# Autodesk Inventor assembly: Box Arm
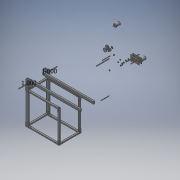
[picture p0: Inventor's stored thumbnail of the model, 180x180]
Saved by Autodesk Inventor 2018 (Build 220112000, 112)
## iProperties
Created: 2019-01-16
Part Number: Box Arm
Document SubType Name: Assembly
Designer: Gabriel
Author: Gabriel
## Documents named in this file (29)
- C:\Users\Gabriel\Documents\GitHub\2019CAD\Drivebase Box Arm\Box Arm.iam
- C:\Users\Gabriel\Documents\GitHub\2019CAD\Drivebase Box Arm\30in 1x1 Beam.ipt
- C:\Users\Gabriel\Documents\GitHub\2019CAD\Drivebase Box Arm\25in 1x1 Beam.ipt
- C:\Users\Gabriel\Documents\GitHub\2019CAD\Drivebase Box Arm\17in 1x1 Beam.ipt
- C:\Users\Gabriel\Documents\GitHub\2019CAD\Drivebase Box Arm\23in 1x1 Beam.ipt
- C:\Users\Gabriel\Documents\GitHub\2019CAD\Drivebase Box Arm\L gusset.ipt
- C:\Users\Gabriel\Documents\GitHub\2019CAD\Drivebase Box Arm\34.48in Arm Bea.ipt
- C:\Users\Gabriel\Documents\GitHub\2019CAD\Drivebase Box Arm\0_500_ID_x_1_125_OD_x_0_313_WD_Flanged_Bearing_217-2731.ipt
- C:\Users\Gabriel\Documents\GitHub\2019CAD\Drivebase Box Arm\_72t_Aluminum_Plate_Sprocket_25_Chain_1-1_8_Bearing_Bore_217-2627.ipt
- C:\Users\Gabriel\Documents\GitHub\2019CAD\Drivebase Box Arm\Hex Hub.ipt
- C:\Users\Gabriel\Documents\GitHub\2019CAD\Drivebase Box Arm\0.5in Hex Shaft.ipt
- C:\Users\Gabriel\Documents\GitHub\2019CAD\Drivebase Box Arm\half_inch_collar.ipt
- C:\Users\Gabriel\Documents\GitHub\2019CAD\Drivebase Box Arm\1_2_Acetal_Spacer_-_1_2_Hex_217-3261.ipt
- C:\Users\Gabriel\Documents\GitHub\2019CAD\Drivebase Box Arm\am-0150 Toughbox Large Output Gear.ipt
- C:\Users\Gabriel\Documents\GitHub\2019CAD\Drivebase Box Arm\Mini_CIM_Motor_217-3371.ipt
- C:\Users\Gabriel\Documents\GitHub\2019CAD\Drivebase Box Arm\ARm Gearbox Plate.ipt
- C:\Users\Gabriel\Documents\GitHub\2019CAD\Drivebase Box Arm\1_16_Acetal_Spacer_-_1_2_Hex_217-3257.ipt
- C:\Users\Gabriel\Documents\GitHub\2019CAD\Drivebase Box Arm\3_8in Hex Shaft.ipt
- C:\Users\Gabriel\Documents\GitHub\2019CAD\Drivebase Box Arm\10T_Steel_Spur_Gear_20_DP_12T_Center_Distance_CIM_Motor_217-6334.ipt
- C:\Users\Gabriel\Documents\GitHub\2019CAD\Drivebase Box Arm\am-0143 50 Tooth 20 dp Aluminum Gear 375 Hex.ipt
- C:\Users\Gabriel\Documents\GitHub\2019CAD\Drivebase Box Arm\am-0151 14T 20dp 375hex.ipt
- C:\Users\Gabriel\Documents\GitHub\2019CAD\Drivebase Box Arm\1_16_Acetal_Spacer_-_3_8_Hex_217-3258.ipt
- C:\Users\Gabriel\Documents\GitHub\2019CAD\Drivebase Box Arm\40t_Aluminum_Spur_Gear_20_DP_3_8_Hex_Bore_217-2707.ipt
- C:\Users\Gabriel\Documents\GitHub\2019CAD\Drivebase Box Arm\am-0028 00.375'' id Flanged, Shielded Ball Bearing (FR6ZZ).ipt
- C:\Users\Gabriel\Documents\GitHub\2019CAD\Drivebase Box Arm\USS flat washer #10 2993.ipt
- C:\Users\Gabriel\Documents\GitHub\2019CAD\Drivebase Box Arm\92196A271_18-8 STAINLESS STEEL SOCKET HEAD CAP SCREW.ipt
- C:\Users\Gabriel\Documents\GitHub\2019CAD\Drivebase Box Arm\am-3621 - S25-18HA-500H.ipt
- C:\Users\Gabriel\Downloads\Clamping_Shaft_Collar_-_1_2_Hex_ID_217-2737.ipt
- C:\Users\Gabriel\Downloads\Clamping_Shaft_Collar_-_3_8_Hex_ID_217-2739.ipt
## Components (108 placed, 28 different names)
1. 30in 1x1 Beam:1 — Mate:13, Mate:14, Mate:37, Mate:38, Mate:74, Mate:75, Mate:83, Mate:84, Mate:98, Mate:99, Mate:101, Mate:102, Mate:103, Mate:104
2. 30in 1x1 Beam:2 — Mate:11, Mate:12, Mate:39, Mate:40, Mate:73, Mate:76, Mate:86, Mate:87, Mate:95, Mate:96, Mate:105, Mate:106, Mate:107, Mate:108
3. 25in 1x1 Beam:1 — Mate:57, Mate:58, Mate:59, Mate:60, Mate:65, Mate:66, Mate:90, Mate:91
4. 25in 1x1 Beam:2 — Mate:61, Mate:62, Mate:63, Mate:64, Mate:67, Mate:68, Mate:93, Mate:94
5. 25in 1x1 Beam:3 — Mate:29, Mate:30, Mate:53, Mate:54, Mate:97
6. 25in 1x1 Beam:4 — Mate:31, Mate:32, Mate:55, Mate:56, Mate:100
7. 17in 1x1 Beam:1 — Mate:69, Mate:70, Mate:71, Mate:72
8. 17in 1x1 Beam:2 — Mate:21, Mate:22, Mate:23, Mate:24
9. 23in 1x1 Beam:1 — Mate:43, Mate:44, Mate:49, Mate:50, Mate:88, Mate:92
10. 23in 1x1 Beam:2 — Mate:47, Mate:48, Mate:51, Mate:52, Mate:85, Mate:89
11. L gusset:1 — Mate:53, Mate:54, Mate:63, Mate:64
12. L gusset:4 — Mate:49, Mate:50, Mate:61, Mate:62
13. L gusset:5 — Mate:51, Mate:52, Mate:57, Mate:58
14. L gusset:7 — Mate:11, Mate:12, Mate:23, Mate:24
15. L gusset:9 — Mate:13, Mate:14, Mate:21, Mate:22
16. L gusset:11 — Mate:31, Mate:32, Mate:74, Mate:75
17. L gusset:12 — Mate:29, Mate:30, Mate:73, Mate:76
18. L gusset:13 — Mate:43, Mate:44
19. L gusset:14 — Mate:47, Mate:48
20. L gusset:15 — Mate:39, Mate:40, Mate:77, Mate:80
21. L gusset:16 — Mate:37, Mate:38, Mate:78, Mate:79
22. L gusset:17 — Mate:55, Mate:56, Mate:59, Mate:60
23. L gusset:18 — Mate:67, Mate:68, Mate:69, Mate:70
24. L gusset:19 — Mate:65, Mate:66, Mate:71, Mate:72
25. 17in 1x1 Beam:3 — Mate:77, Mate:78, Mate:79, Mate:80
26. 34.48in Arm Bea:2 — Mate:109, Mate:110
27. 0_500_ID_x_1_125_OD_x_0_313_WD_Flanged_Bearing_217-2731:1 — Mate:103, Mate:104, Mate:139, Mate:140, Mate:149
28. 0_500_ID_x_1_125_OD_x_0_313_WD_Flanged_Bearing_217-2731:2 — Mate:107, Mate:108, Mate:126, Mate:152
29. 0_500_ID_x_1_125_OD_x_0_313_WD_Flanged_Bearing_217-2731:5 — Mate:101, Mate:102, Mate:143
30. 0_500_ID_x_1_125_OD_x_0_313_WD_Flanged_Bearing_217-2731:8 — Mate:105, Mate:106, Mate:122
31. L gusset:20 — Mate:92, Mate:93, Mate:94
32. L gusset:21 — Mate:89, Mate:90, Mate:91
33. L gusset:22 — Mate:98, Mate:99, Mate:100
34. L gusset:23 — Mate:95, Mate:96, Mate:97
35. L gusset:24 — Mate:83, Mate:84, Mate:85
36. L gusset:25 — Mate:86, Mate:87, Mate:88
37. _72t_Aluminum_Plate_Sprocket_25_Chain_1-1_8_Bearing_Bore_217-2627:2 — Mate:120, Mate:121, Mate:138
38. Hex Hub:2 — Mate:109, Mate:110, Mate:111, Mate:112, Mate:113, Mate:114, Mate:115
39. Hex Hub:3 — Mate:116, Mate:117, Mate:118, Mate:120, Mate:121, Mate:122, Mate:138
40. 0.5in Hex Shaft:2 — Mate:114, Mate:115, Mate:116, Mate:117, Mate:123, Mate:124, Mate:125, Mate:150, Mate:151, Mate:404, Mate:405
41. 1_2_Acetal_Spacer_-_1_2_Hex_217-3261:1 — Mate:123, Mate:124, Mate:125, Mate:126, Mate:406
42. 1_2_Acetal_Spacer_-_1_2_Hex_217-3261:3 — Mate:111, Mate:112, Mate:113, Mate:118
43. 34.48in Arm Bea:3 — Mate:128
44. _72t_Aluminum_Plate_Sprocket_25_Chain_1-1_8_Bearing_Bore_217-2627:3 — Mate:137
45. Hex Hub:4 — Mate:134, Mate:135, Mate:136, Mate:137, Mate:139, Mate:140
46. Hex Hub:5 — Mate:128, Mate:129, Mate:130, Mate:133
47. 0.5in Hex Shaft:3 — Mate:129, Mate:130, Mate:131, Mate:132, Mate:134, Mate:135, Mate:141, Mate:142, Mate:147, Mate:148, Mate:401, Mate:402
48. 1_2_Acetal_Spacer_-_1_2_Hex_217-3261:7 — Mate:141, Mate:142, Mate:143, Mate:403
49. 1_2_Acetal_Spacer_-_1_2_Hex_217-3261:8 — Mate:131, Mate:132, Mate:133, Mate:136
50. 1_2_Acetal_Spacer_-_1_2_Hex_217-3261:9 — Mate:147, Mate:148, Mate:149
51. 1_2_Acetal_Spacer_-_1_2_Hex_217-3261:10 — Mate:150, Mate:151, Mate:152
52. 0.5in Hex Shaft:4
53. 0.5in Hex Shaft:5 — Mate:345, Mate:346, Mate:347, Mate:348, Mate:349, Mate:350, Mate:351, Mate:370, Mate:371, Mate:386, Mate:387, Mate:389, Mate:390, Mate:395, Mate:396, Mate:398, Mate:399
54. half_inch_collar:9
55. Mini_CIM_Motor_217-3371:5 — Mate:368, Mate:369, Mate:374
56. am-0150 Toughbox Large Output Gear:8 — Mate:345, Mate:346, Mate:347, Mate:352
57. Mini_CIM_Motor_217-3371:8
58. 1_16_Acetal_Spacer_-_1_2_Hex_217-3257:4 — Mate:348, Mate:349, Mate:352, Mate:353
59. 1_16_Acetal_Spacer_-_1_2_Hex_217-3257:6 — Mate:350, Mate:351, Mate:353, Mate:354
60. 1_16_Acetal_Spacer_-_1_2_Hex_217-3257:8 — Mate:370, Mate:371, Mate:372, Mate:388
61. 3_8in Hex Shaft:2
62. 3_8in Hex Shaft:5 — Mate:313, Mate:314, Mate:315, Mate:316, Mate:317, Mate:318, Mate:321, Mate:322, Mate:357, Mate:358, Mate:394
63. am-0151 14T 20dp 375hex:1 — Mate:325, Mate:326, Mate:331, Mate:335
64. am-0151 14T 20dp 375hex:3 — Mate:315, Mate:316, Mate:320, Mate:359
65. 10T_Steel_Spur_Gear_20_DP_12T_Center_Distance_CIM_Motor_217-6334:4
66. am-0151 14T 20dp 375hex:4
67. am-0143 50 Tooth 20 dp Aluminum Gear 375 Hex:5 — Mate:327, Mate:328, Mate:332, Mate:339
68. 10T_Steel_Spur_Gear_20_DP_12T_Center_Distance_CIM_Motor_217-6334:6 — Mate:374
69. am-0143 50 Tooth 20 dp Aluminum Gear 375 Hex:6
70. am-0151 14T 20dp 375hex:6
71. 1_16_Acetal_Spacer_-_3_8_Hex_217-3258:2 — Mate:337, Mate:338, Mate:339
72. 1_16_Acetal_Spacer_-_3_8_Hex_217-3258:3 — Mate:333, Mate:334, Mate:335, Mate:384
73. 1_16_Acetal_Spacer_-_3_8_Hex_217-3258:5 — Mate:321, Mate:322, Mate:323
74. 1_16_Acetal_Spacer_-_3_8_Hex_217-3258:6 — Mate:317, Mate:318, Mate:319, Mate:320
75. 40t_Aluminum_Spur_Gear_20_DP_3_8_Hex_Bore_217-2707:1 — Mate:313, Mate:314, Mate:319, Mate:323
76. 40t_Aluminum_Spur_Gear_20_DP_3_8_Hex_Bore_217-2707:3
77. 3_8in Hex Shaft:8
78. 3_8in Hex Shaft:10 — Mate:325, Mate:326, Mate:327, Mate:328, Mate:329, Mate:330, Mate:333, Mate:334, Mate:337, Mate:338
79. ARm Gearbox Plate:5 — Mate:341, Mate:344, Mate:378, Mate:379, Mate:382, Mate:383
80. ARm Gearbox Plate:6 — Mate:342, Mate:343, Mate:360, Mate:361, Mate:362, Mate:363, Mate:365, Mate:367, Mate:376, Mate:377, Mate:380, Mate:381
81. 1_16_Acetal_Spacer_-_3_8_Hex_217-3258:8 — Mate:357, Mate:358, Mate:359
82. 1_16_Acetal_Spacer_-_3_8_Hex_217-3258:10 — Mate:329, Mate:330, Mate:331, Mate:332
83. 0_500_ID_x_1_125_OD_x_0_313_WD_Flanged_Bearing_217-2731:9 — Mate:341, Mate:344, Mate:400
84. 0_500_ID_x_1_125_OD_x_0_313_WD_Flanged_Bearing_217-2731:10 — Mate:342, Mate:343, Mate:354, Mate:372
85. USS flat washer #10 2993:1 — Mate:366, Mate:367, Mate:369
86. USS flat washer #10 2993:2 — Mate:364, Mate:365
87. 92196A271_18-8 STAINLESS STEEL SOCKET HEAD CAP SCREW:1 — Mate:361, Mate:363, Mate:366
88. 92196A271_18-8 STAINLESS STEEL SOCKET HEAD CAP SCREW:2 — Mate:360, Mate:362, Mate:364, Mate:368
89. am-0028 00.375'' id Flanged, Shielded Ball Bearing (FR6ZZ):2 — Mate:376, Mate:380, Mate:384
90. am-0028 00.375'' id Flanged, Shielded Ball Bearing (FR6ZZ):3 — Mate:378, Mate:383
91. am-0028 00.375'' id Flanged, Shielded Ball Bearing (FR6ZZ):4 — Mate:379, Mate:382
92. am-0028 00.375'' id Flanged, Shielded Ball Bearing (FR6ZZ):5 — Mate:377, Mate:381, Mate:394
93. am-0150 Toughbox Large Output Gear:9
94. am-3621 - S25-18HA-500H:1 — Mate:386, Mate:387, Mate:388, Mate:391
95. 1_2_Acetal_Spacer_-_1_2_Hex_217-3261:11 — Mate:389, Mate:390, Mate:391, Mate:397
96. am-3621 - S25-18HA-500H:2
97. Clamping_Shaft_Collar_-_1_2_Hex_ID_217-2737:1 — Mate:395, Mate:396, Mate:397
98. Clamping_Shaft_Collar_-_3_8_Hex_ID_217-2739:1
99. Clamping_Shaft_Collar_-_1_2_Hex_ID_217-2737:2 — Mate:398, Mate:399, Mate:400
100. Clamping_Shaft_Collar_-_3_8_Hex_ID_217-2739:2
101. Clamping_Shaft_Collar_-_1_2_Hex_ID_217-2737:3
102. Clamping_Shaft_Collar_-_3_8_Hex_ID_217-2739:3
103. Clamping_Shaft_Collar_-_1_2_Hex_ID_217-2737:4
104. Clamping_Shaft_Collar_-_3_8_Hex_ID_217-2739:4
105. Clamping_Shaft_Collar_-_1_2_Hex_ID_217-2737:5 — Mate:404, Mate:405, Mate:406
106. Clamping_Shaft_Collar_-_3_8_Hex_ID_217-2739:5
107. Clamping_Shaft_Collar_-_1_2_Hex_ID_217-2737:6 — Mate:401, Mate:402, Mate:403
108. Clamping_Shaft_Collar_-_3_8_Hex_ID_217-2739:6
## Relationships (201: Mate 201)
- Mate:11: 30in 1x1 Beam:2 ↔ L gusset:7
- Mate:12: 30in 1x1 Beam:2 ↔ L gusset:7
- Mate:13: 30in 1x1 Beam:1 ↔ L gusset:9
- Mate:14: 30in 1x1 Beam:1 ↔ L gusset:9
- Mate:21: 17in 1x1 Beam:2 ↔ L gusset:9
- Mate:22: 17in 1x1 Beam:2 ↔ L gusset:9
- Mate:23: 17in 1x1 Beam:2 ↔ L gusset:7
- Mate:24: 17in 1x1 Beam:2 ↔ L gusset:7
- Mate:29: 25in 1x1 Beam:3 ↔ L gusset:12
- Mate:30: 25in 1x1 Beam:3 ↔ L gusset:12
- Mate:31: 25in 1x1 Beam:4 ↔ L gusset:11
- Mate:32: 25in 1x1 Beam:4 ↔ L gusset:11
- Mate:37: 30in 1x1 Beam:1 ↔ L gusset:16
- Mate:38: 30in 1x1 Beam:1 ↔ L gusset:16
- Mate:39: 30in 1x1 Beam:2 ↔ L gusset:15
- Mate:40: 30in 1x1 Beam:2 ↔ L gusset:15
- Mate:43: 23in 1x1 Beam:1 ↔ L gusset:13
- Mate:44: 23in 1x1 Beam:1 ↔ L gusset:13
- Mate:47: 23in 1x1 Beam:2 ↔ L gusset:14
- Mate:48: 23in 1x1 Beam:2 ↔ L gusset:14
- Mate:49: 23in 1x1 Beam:1 ↔ L gusset:4
- Mate:50: 23in 1x1 Beam:1 ↔ L gusset:4
- Mate:51: 23in 1x1 Beam:2 ↔ L gusset:5
- Mate:52: 23in 1x1 Beam:2 ↔ L gusset:5
- Mate:53: 25in 1x1 Beam:3 ↔ L gusset:1
- Mate:54: 25in 1x1 Beam:3 ↔ L gusset:1
- Mate:55: 25in 1x1 Beam:4 ↔ L gusset:17
- Mate:56: 25in 1x1 Beam:4 ↔ L gusset:17
- Mate:57: 25in 1x1 Beam:1 ↔ L gusset:5
- Mate:58: 25in 1x1 Beam:1 ↔ L gusset:5
- Mate:59: 25in 1x1 Beam:1 ↔ L gusset:17
- Mate:60: 25in 1x1 Beam:1 ↔ L gusset:17
- Mate:61: 25in 1x1 Beam:2 ↔ L gusset:4
- Mate:62: 25in 1x1 Beam:2 ↔ L gusset:4
- Mate:63: 25in 1x1 Beam:2 ↔ L gusset:1
- Mate:64: 25in 1x1 Beam:2 ↔ L gusset:1
- Mate:65: 25in 1x1 Beam:1 ↔ L gusset:19
- Mate:66: 25in 1x1 Beam:1 ↔ L gusset:19
- Mate:67: 25in 1x1 Beam:2 ↔ L gusset:18
- Mate:68: 25in 1x1 Beam:2 ↔ L gusset:18
- Mate:69: 17in 1x1 Beam:1 ↔ L gusset:18
- Mate:70: 17in 1x1 Beam:1 ↔ L gusset:18
- Mate:71: 17in 1x1 Beam:1 ↔ L gusset:19
- Mate:72: 17in 1x1 Beam:1 ↔ L gusset:19
- Mate:73: 30in 1x1 Beam:2 ↔ L gusset:12
- Mate:74: 30in 1x1 Beam:1 ↔ L gusset:11
- Mate:75: 30in 1x1 Beam:1 ↔ L gusset:11
- Mate:76: 30in 1x1 Beam:2 ↔ L gusset:12
- Mate:77: L gusset:15 ↔ 17in 1x1 Beam:3
- Mate:78: L gusset:16 ↔ 17in 1x1 Beam:3
- Mate:79: L gusset:16 ↔ 17in 1x1 Beam:3
- Mate:80: L gusset:15 ↔ 17in 1x1 Beam:3
- Mate:83: 30in 1x1 Beam:1 ↔ L gusset:24
- Mate:84: 30in 1x1 Beam:1 ↔ L gusset:24
- Mate:85: 23in 1x1 Beam:2 ↔ L gusset:24
- Mate:86: 30in 1x1 Beam:2 ↔ L gusset:25
- Mate:87: 30in 1x1 Beam:2 ↔ L gusset:25
- Mate:88: 23in 1x1 Beam:1 ↔ L gusset:25
- Mate:89: 23in 1x1 Beam:2 ↔ L gusset:21
- Mate:90: 25in 1x1 Beam:1 ↔ L gusset:21
- Mate:91: 25in 1x1 Beam:1 ↔ L gusset:21
- Mate:92: 23in 1x1 Beam:1 ↔ L gusset:20
- Mate:93: 25in 1x1 Beam:2 ↔ L gusset:20
- Mate:94: 25in 1x1 Beam:2 ↔ L gusset:20
- Mate:95: 30in 1x1 Beam:2 ↔ L gusset:23
- Mate:96: 30in 1x1 Beam:2 ↔ L gusset:23
- Mate:97: 25in 1x1 Beam:3 ↔ L gusset:23
- Mate:98: 30in 1x1 Beam:1 ↔ L gusset:22
- Mate:99: 30in 1x1 Beam:1 ↔ L gusset:22
- Mate:100: 25in 1x1 Beam:4 ↔ L gusset:22
- Mate:101: 30in 1x1 Beam:1 ↔ 0_500_ID_x_1_125_OD_x_0_313_WD_Flanged_Bearing_217-2731:5
- Mate:102: 30in 1x1 Beam:1 ↔ 0_500_ID_x_1_125_OD_x_0_313_WD_Flanged_Bearing_217-2731:5
- Mate:103: 30in 1x1 Beam:1 ↔ 0_500_ID_x_1_125_OD_x_0_313_WD_Flanged_Bearing_217-2731:1
- Mate:104: 30in 1x1 Beam:1 ↔ 0_500_ID_x_1_125_OD_x_0_313_WD_Flanged_Bearing_217-2731:1
- Mate:105: 30in 1x1 Beam:2 ↔ 0_500_ID_x_1_125_OD_x_0_313_WD_Flanged_Bearing_217-2731:8
- Mate:106: 30in 1x1 Beam:2 ↔ 0_500_ID_x_1_125_OD_x_0_313_WD_Flanged_Bearing_217-2731:8
- Mate:107: 30in 1x1 Beam:2 ↔ 0_500_ID_x_1_125_OD_x_0_313_WD_Flanged_Bearing_217-2731:2
- Mate:108: 30in 1x1 Beam:2 ↔ 0_500_ID_x_1_125_OD_x_0_313_WD_Flanged_Bearing_217-2731:2
- Mate:109: 34.48in Arm Bea:2 ↔ Hex Hub:2
- Mate:110: 34.48in Arm Bea:2 ↔ Hex Hub:2
- Mate:111: Hex Hub:2 ↔ 1_2_Acetal_Spacer_-_1_2_Hex_217-3261:3
- Mate:112: Hex Hub:2 ↔ 1_2_Acetal_Spacer_-_1_2_Hex_217-3261:3
- Mate:113: Hex Hub:2 ↔ 1_2_Acetal_Spacer_-_1_2_Hex_217-3261:3
- Mate:114: Hex Hub:2 ↔ 0.5in Hex Shaft:2
- Mate:115: Hex Hub:2 ↔ 0.5in Hex Shaft:2
- Mate:116: Hex Hub:3 ↔ 0.5in Hex Shaft:2
- Mate:117: Hex Hub:3 ↔ 0.5in Hex Shaft:2
- Mate:118: Hex Hub:3 ↔ 1_2_Acetal_Spacer_-_1_2_Hex_217-3261:3
- Mate:120: _72t_Aluminum_Plate_Sprocket_25_Chain_1-1_8_Bearing_Bore_217-2627:2 ↔ Hex Hub:3
- Mate:121: _72t_Aluminum_Plate_Sprocket_25_Chain_1-1_8_Bearing_Bore_217-2627:2 ↔ Hex Hub:3
- Mate:122: 0_500_ID_x_1_125_OD_x_0_313_WD_Flanged_Bearing_217-2731:8 ↔ Hex Hub:3
- Mate:123: 0.5in Hex Shaft:2 ↔ 1_2_Acetal_Spacer_-_1_2_Hex_217-3261:1
- Mate:124: 0.5in Hex Shaft:2 ↔ 1_2_Acetal_Spacer_-_1_2_Hex_217-3261:1
- Mate:125: 0.5in Hex Shaft:2 ↔ 1_2_Acetal_Spacer_-_1_2_Hex_217-3261:1
- Mate:126: 0_500_ID_x_1_125_OD_x_0_313_WD_Flanged_Bearing_217-2731:2 ↔ 1_2_Acetal_Spacer_-_1_2_Hex_217-3261:1
- Mate:128: 34.48in Arm Bea:3 ↔ Hex Hub:5
- Mate:129: Hex Hub:5 ↔ 0.5in Hex Shaft:3
- Mate:130: Hex Hub:5 ↔ 0.5in Hex Shaft:3
- Mate:131: 0.5in Hex Shaft:3 ↔ 1_2_Acetal_Spacer_-_1_2_Hex_217-3261:8
- Mate:132: 0.5in Hex Shaft:3 ↔ 1_2_Acetal_Spacer_-_1_2_Hex_217-3261:8
- Mate:133: Hex Hub:5 ↔ 1_2_Acetal_Spacer_-_1_2_Hex_217-3261:8
- Mate:134: Hex Hub:4 ↔ 0.5in Hex Shaft:3
- Mate:135: Hex Hub:4 ↔ 0.5in Hex Shaft:3
- Mate:136: Hex Hub:4 ↔ 1_2_Acetal_Spacer_-_1_2_Hex_217-3261:8
- Mate:137: _72t_Aluminum_Plate_Sprocket_25_Chain_1-1_8_Bearing_Bore_217-2627:3 ↔ Hex Hub:4
- Mate:138: _72t_Aluminum_Plate_Sprocket_25_Chain_1-1_8_Bearing_Bore_217-2627:2 ↔ Hex Hub:3
- Mate:139: 0_500_ID_x_1_125_OD_x_0_313_WD_Flanged_Bearing_217-2731:1 ↔ Hex Hub:4
- Mate:140: 0_500_ID_x_1_125_OD_x_0_313_WD_Flanged_Bearing_217-2731:1 ↔ Hex Hub:4
- Mate:141: 0.5in Hex Shaft:3 ↔ 1_2_Acetal_Spacer_-_1_2_Hex_217-3261:7
- Mate:142: 0.5in Hex Shaft:3 ↔ 1_2_Acetal_Spacer_-_1_2_Hex_217-3261:7
- Mate:143: 0_500_ID_x_1_125_OD_x_0_313_WD_Flanged_Bearing_217-2731:5 ↔ 1_2_Acetal_Spacer_-_1_2_Hex_217-3261:7
- Mate:147: 0.5in Hex Shaft:3 ↔ 1_2_Acetal_Spacer_-_1_2_Hex_217-3261:9
- Mate:148: 0.5in Hex Shaft:3 ↔ 1_2_Acetal_Spacer_-_1_2_Hex_217-3261:9
- Mate:149: 0_500_ID_x_1_125_OD_x_0_313_WD_Flanged_Bearing_217-2731:1 ↔ 1_2_Acetal_Spacer_-_1_2_Hex_217-3261:9
- Mate:150: 0.5in Hex Shaft:2 ↔ 1_2_Acetal_Spacer_-_1_2_Hex_217-3261:10
- Mate:151: 0.5in Hex Shaft:2 ↔ 1_2_Acetal_Spacer_-_1_2_Hex_217-3261:10
- Mate:152: 0_500_ID_x_1_125_OD_x_0_313_WD_Flanged_Bearing_217-2731:2 ↔ 1_2_Acetal_Spacer_-_1_2_Hex_217-3261:10
- Mate:313: 3_8in Hex Shaft:5 ↔ 40t_Aluminum_Spur_Gear_20_DP_3_8_Hex_Bore_217-2707:1
- Mate:314: 3_8in Hex Shaft:5 ↔ 40t_Aluminum_Spur_Gear_20_DP_3_8_Hex_Bore_217-2707:1
- Mate:315: 3_8in Hex Shaft:5 ↔ am-0151 14T 20dp 375hex:3
- Mate:316: 3_8in Hex Shaft:5 ↔ am-0151 14T 20dp 375hex:3
- Mate:317: 3_8in Hex Shaft:5 ↔ 1_16_Acetal_Spacer_-_3_8_Hex_217-3258:6
- Mate:318: 3_8in Hex Shaft:5 ↔ 1_16_Acetal_Spacer_-_3_8_Hex_217-3258:6
- Mate:319: 1_16_Acetal_Spacer_-_3_8_Hex_217-3258:6 ↔ 40t_Aluminum_Spur_Gear_20_DP_3_8_Hex_Bore_217-2707:1
- Mate:320: am-0151 14T 20dp 375hex:3 ↔ 1_16_Acetal_Spacer_-_3_8_Hex_217-3258:6
- Mate:321: 3_8in Hex Shaft:5 ↔ 1_16_Acetal_Spacer_-_3_8_Hex_217-3258:5
- Mate:322: 3_8in Hex Shaft:5 ↔ 1_16_Acetal_Spacer_-_3_8_Hex_217-3258:5
- Mate:323: 1_16_Acetal_Spacer_-_3_8_Hex_217-3258:5 ↔ 40t_Aluminum_Spur_Gear_20_DP_3_8_Hex_Bore_217-2707:1
- Mate:325: am-0151 14T 20dp 375hex:1 ↔ 3_8in Hex Shaft:10
- Mate:326: am-0151 14T 20dp 375hex:1 ↔ 3_8in Hex Shaft:10
- Mate:327: am-0143 50 Tooth 20 dp Aluminum Gear 375 Hex:5 ↔ 3_8in Hex Shaft:10
- Mate:328: am-0143 50 Tooth 20 dp Aluminum Gear 375 Hex:5 ↔ 3_8in Hex Shaft:10
- Mate:329: 3_8in Hex Shaft:10 ↔ 1_16_Acetal_Spacer_-_3_8_Hex_217-3258:10
- Mate:330: 3_8in Hex Shaft:10 ↔ 1_16_Acetal_Spacer_-_3_8_Hex_217-3258:10
- Mate:331: am-0151 14T 20dp 375hex:1 ↔ 1_16_Acetal_Spacer_-_3_8_Hex_217-3258:10
- Mate:332: am-0143 50 Tooth 20 dp Aluminum Gear 375 Hex:5 ↔ 1_16_Acetal_Spacer_-_3_8_Hex_217-3258:10
- Mate:333: 1_16_Acetal_Spacer_-_3_8_Hex_217-3258:3 ↔ 3_8in Hex Shaft:10
- Mate:334: 1_16_Acetal_Spacer_-_3_8_Hex_217-3258:3 ↔ 3_8in Hex Shaft:10
- Mate:335: am-0151 14T 20dp 375hex:1 ↔ 1_16_Acetal_Spacer_-_3_8_Hex_217-3258:3
- Mate:337: 1_16_Acetal_Spacer_-_3_8_Hex_217-3258:2 ↔ 3_8in Hex Shaft:10
- Mate:338: 1_16_Acetal_Spacer_-_3_8_Hex_217-3258:2 ↔ 3_8in Hex Shaft:10
- Mate:339: am-0143 50 Tooth 20 dp Aluminum Gear 375 Hex:5 ↔ 1_16_Acetal_Spacer_-_3_8_Hex_217-3258:2
- Mate:341: ARm Gearbox Plate:5 ↔ 0_500_ID_x_1_125_OD_x_0_313_WD_Flanged_Bearing_217-2731:9
- Mate:342: ARm Gearbox Plate:6 ↔ 0_500_ID_x_1_125_OD_x_0_313_WD_Flanged_Bearing_217-2731:10
- Mate:343: ARm Gearbox Plate:6 ↔ 0_500_ID_x_1_125_OD_x_0_313_WD_Flanged_Bearing_217-2731:10
- Mate:344: ARm Gearbox Plate:5 ↔ 0_500_ID_x_1_125_OD_x_0_313_WD_Flanged_Bearing_217-2731:9
- Mate:345: 0.5in Hex Shaft:5 ↔ am-0150 Toughbox Large Output Gear:8
- Mate:346: 0.5in Hex Shaft:5 ↔ am-0150 Toughbox Large Output Gear:8
- Mate:347: 0.5in Hex Shaft:5 ↔ am-0150 Toughbox Large Output Gear:8
- Mate:348: 0.5in Hex Shaft:5 ↔ 1_16_Acetal_Spacer_-_1_2_Hex_217-3257:4
- Mate:349: 0.5in Hex Shaft:5 ↔ 1_16_Acetal_Spacer_-_1_2_Hex_217-3257:4
- Mate:350: 0.5in Hex Shaft:5 ↔ 1_16_Acetal_Spacer_-_1_2_Hex_217-3257:6
- Mate:351: 0.5in Hex Shaft:5 ↔ 1_16_Acetal_Spacer_-_1_2_Hex_217-3257:6
- Mate:352: am-0150 Toughbox Large Output Gear:8 ↔ 1_16_Acetal_Spacer_-_1_2_Hex_217-3257:4
- Mate:353: 1_16_Acetal_Spacer_-_1_2_Hex_217-3257:4 ↔ 1_16_Acetal_Spacer_-_1_2_Hex_217-3257:6
- Mate:354: 1_16_Acetal_Spacer_-_1_2_Hex_217-3257:6 ↔ 0_500_ID_x_1_125_OD_x_0_313_WD_Flanged_Bearing_217-2731:10
- Mate:357: 3_8in Hex Shaft:5 ↔ 1_16_Acetal_Spacer_-_3_8_Hex_217-3258:8
- Mate:358: 3_8in Hex Shaft:5 ↔ 1_16_Acetal_Spacer_-_3_8_Hex_217-3258:8
- Mate:359: am-0151 14T 20dp 375hex:3 ↔ 1_16_Acetal_Spacer_-_3_8_Hex_217-3258:8
- Mate:360: ARm Gearbox Plate:6 ↔ 92196A271_18-8 STAINLESS STEEL SOCKET HEAD CAP SCREW:2
- Mate:361: ARm Gearbox Plate:6 ↔ 92196A271_18-8 STAINLESS STEEL SOCKET HEAD CAP SCREW:1
- Mate:362: ARm Gearbox Plate:6 ↔ 92196A271_18-8 STAINLESS STEEL SOCKET HEAD CAP SCREW:2
- Mate:363: ARm Gearbox Plate:6 ↔ 92196A271_18-8 STAINLESS STEEL SOCKET HEAD CAP SCREW:1
- Mate:364: USS flat washer #10 2993:2 ↔ 92196A271_18-8 STAINLESS STEEL SOCKET HEAD CAP SCREW:2
- Mate:365: ARm Gearbox Plate:6 ↔ USS flat washer #10 2993:2
- Mate:366: USS flat washer #10 2993:1 ↔ 92196A271_18-8 STAINLESS STEEL SOCKET HEAD CAP SCREW:1
- Mate:367: ARm Gearbox Plate:6 ↔ USS flat washer #10 2993:1
- Mate:368: Mini_CIM_Motor_217-3371:5 ↔ 92196A271_18-8 STAINLESS STEEL SOCKET HEAD CAP SCREW:2
- Mate:369: Mini_CIM_Motor_217-3371:5 ↔ USS flat washer #10 2993:1
- Mate:370: 0.5in Hex Shaft:5 ↔ 1_16_Acetal_Spacer_-_1_2_Hex_217-3257:8
- Mate:371: 0.5in Hex Shaft:5 ↔ 1_16_Acetal_Spacer_-_1_2_Hex_217-3257:8
- Mate:372: 1_16_Acetal_Spacer_-_1_2_Hex_217-3257:8 ↔ 0_500_ID_x_1_125_OD_x_0_313_WD_Flanged_Bearing_217-2731:10
- Mate:374: Mini_CIM_Motor_217-3371:5 ↔ 10T_Steel_Spur_Gear_20_DP_12T_Center_Distance_CIM_Motor_217-6334:6
- Mate:376: ARm Gearbox Plate:6 ↔ am-0028 00.375'' id Flanged, Shielded Ball Bearing (FR6ZZ):2
- Mate:377: ARm Gearbox Plate:6 ↔ am-0028 00.375'' id Flanged, Shielded Ball Bearing (FR6ZZ):5
- Mate:378: ARm Gearbox Plate:5 ↔ am-0028 00.375'' id Flanged, Shielded Ball Bearing (FR6ZZ):3
- Mate:379: ARm Gearbox Plate:5 ↔ am-0028 00.375'' id Flanged, Shielded Ball Bearing (FR6ZZ):4
- Mate:380: ARm Gearbox Plate:6 ↔ am-0028 00.375'' id Flanged, Shielded Ball Bearing (FR6ZZ):2
- Mate:381: ARm Gearbox Plate:6 ↔ am-0028 00.375'' id Flanged, Shielded Ball Bearing (FR6ZZ):5
- Mate:382: ARm Gearbox Plate:5 ↔ am-0028 00.375'' id Flanged, Shielded Ball Bearing (FR6ZZ):4
- Mate:383: ARm Gearbox Plate:5 ↔ am-0028 00.375'' id Flanged, Shielded Ball Bearing (FR6ZZ):3
- Mate:384: 1_16_Acetal_Spacer_-_3_8_Hex_217-3258:3 ↔ am-0028 00.375'' id Flanged, Shielded Ball Bearing (FR6ZZ):2
- Mate:386: 0.5in Hex Shaft:5 ↔ am-3621 - S25-18HA-500H:1
- Mate:387: 0.5in Hex Shaft:5 ↔ am-3621 - S25-18HA-500H:1
- Mate:388: 1_16_Acetal_Spacer_-_1_2_Hex_217-3257:8 ↔ am-3621 - S25-18HA-500H:1
- Mate:389: 0.5in Hex Shaft:5 ↔ 1_2_Acetal_Spacer_-_1_2_Hex_217-3261:11
- Mate:390: 0.5in Hex Shaft:5 ↔ 1_2_Acetal_Spacer_-_1_2_Hex_217-3261:11
- Mate:391: am-3621 - S25-18HA-500H:1 ↔ 1_2_Acetal_Spacer_-_1_2_Hex_217-3261:11
- Mate:394: 3_8in Hex Shaft:5 ↔ am-0028 00.375'' id Flanged, Shielded Ball Bearing (FR6ZZ):5
- Mate:395: 0.5in Hex Shaft:5 ↔ Clamping_Shaft_Collar_-_1_2_Hex_ID_217-2737:1
- Mate:396: 0.5in Hex Shaft:5 ↔ Clamping_Shaft_Collar_-_1_2_Hex_ID_217-2737:1
- Mate:397: 1_2_Acetal_Spacer_-_1_2_Hex_217-3261:11 ↔ Clamping_Shaft_Collar_-_1_2_Hex_ID_217-2737:1
- Mate:398: 0.5in Hex Shaft:5 ↔ Clamping_Shaft_Collar_-_1_2_Hex_ID_217-2737:2
- Mate:399: 0.5in Hex Shaft:5 ↔ Clamping_Shaft_Collar_-_1_2_Hex_ID_217-2737:2
- Mate:400: 0_500_ID_x_1_125_OD_x_0_313_WD_Flanged_Bearing_217-2731:9 ↔ Clamping_Shaft_Collar_-_1_2_Hex_ID_217-2737:2
- Mate:401: 0.5in Hex Shaft:3 ↔ Clamping_Shaft_Collar_-_1_2_Hex_ID_217-2737:6
- Mate:402: 0.5in Hex Shaft:3 ↔ Clamping_Shaft_Collar_-_1_2_Hex_ID_217-2737:6
- Mate:403: 1_2_Acetal_Spacer_-_1_2_Hex_217-3261:7 ↔ Clamping_Shaft_Collar_-_1_2_Hex_ID_217-2737:6
- Mate:404: 0.5in Hex Shaft:2 ↔ Clamping_Shaft_Collar_-_1_2_Hex_ID_217-2737:5
- Mate:405: 0.5in Hex Shaft:2 ↔ Clamping_Shaft_Collar_-_1_2_Hex_ID_217-2737:5
- Mate:406: 1_2_Acetal_Spacer_-_1_2_Hex_217-3261:1 ↔ Clamping_Shaft_Collar_-_1_2_Hex_ID_217-2737:5
